# Autodesk Inventor assembly: AM14U3 Square Frame Half
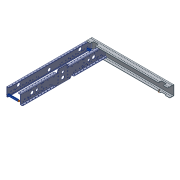
[picture p0: Inventor's stored thumbnail of the model, 180x180]
Saved by Autodesk Inventor 2016 (Build 200138000, 138)
## iProperties
Created: 2016-01-27
Part Number: AM14U3 Square Frame Half
Document SubType Name: Assembly
Designer: PrashantBIA
Author: PrashantBIA
Revision Number: ANY
## Documents named in this file (8)
- C:\Users\PrashantBIA\Desktop\Robotics\Robot Assembly 1-27-15 New Swami\Robot Assembly\Drive Train\AM14U3 Square Frame Half.iam
- C:\Users\PrashantBIA\Desktop\Robotics\Robot Assembly 1-27-15 New Swami\Robot Assembly\Drive Train\FHTS 0.25-20-0.75_FHTS 0.25-20-G-0.75-C.ipt
- C:\Users\PrashantBIA\Desktop\Robotics\Robot Assembly 1-27-15 New Swami\Robot Assembly\Drive Train\Churro 3375.ipt
- C:\Users\PrashantBIA\Desktop\Robotics\Robot Assembly 1-27-15 New Swami\Robot Assembly\Drive Train\10-32x0500_shcs_HX-SHCS 0.19-32x1.375x1-C.ipt
- C:\Users\PrashantBIA\Desktop\Robotics\Robot Assembly 1-27-15 New Swami\Robot Assembly\Drive Train\10-32 Nylock Nut.ipt
- C:\Users\PrashantBIA\Desktop\Robotics\Robot Assembly 1-27-15 New Swami\Robot Assembly\Drive Train\AM14U3 End Sheet Square.ipt
- C:\Users\PrashantBIA\Desktop\Robotics\Robot Assembly 1-27-15 New Swami\Robot Assembly\Drive Train\AM14U3 Inside Sheet Square.ipt
- C:\Users\PrashantBIA\Desktop\Robotics\Robot Assembly 1-27-15 New Swami\Robot Assembly\Drive Train\AM14U3 Outside Sheet Square.ipt
## Components (13 placed, 13 different names)
1. FHTS 0.25-20-0.75_FHTS 0.25-20-G-0.75-C_80
2. FHTS 0.25-20-0.75_FHTS 0.25-20-G-0.75-C_81
3. FHTS 0.25-20-0.75_FHTS 0.25-20-G-0.75-C_82
4. FHTS 0.25-20-0.75_FHTS 0.25-20-G-0.75-C_84
5. Churro 3375_86
6. Churro 3375_87
7. 10-32x0500_shcs_HX-SHCS 0.19-32x1.375x1-C_93
8. 10-32x0500_shcs_HX-SHCS 0.19-32x1.375x1-C_98
9. 10-32 Nylock Nut_107
10. 10-32 Nylock Nut_108
11. AM14U3 End Sheet Square_125 — Mate:3, Mate:4, Mate:5
12. AM14U3 Inside Sheet Square_126 — Mate:1, Flush:1, Flush:2
13. AM14U3 Outside Sheet Square_127 — Mate:1, Flush:1, Flush:2, Mate:3, Mate:4, Mate:5
## Relationships (6: Mate 4, Flush 2)
- Mate:1 (111.125 mm): AM14U3 Inside Sheet Square_126 ↔ AM14U3 Outside Sheet Square_127
- Flush:1: AM14U3 Inside Sheet Square_126 ↔ AM14U3 Outside Sheet Square_127
- Flush:2: AM14U3 Inside Sheet Square_126 ↔ AM14U3 Outside Sheet Square_127
- Mate:3: AM14U3 End Sheet Square_125 ↔ AM14U3 Outside Sheet Square_127
- Mate:4: AM14U3 End Sheet Square_125 ↔ AM14U3 Outside Sheet Square_127
- Mate:5: AM14U3 End Sheet Square_125 ↔ AM14U3 Outside Sheet Square_127
